# Autodesk Inventor assembly: engine moving
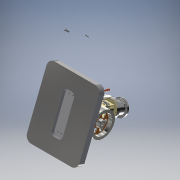
[picture p0: Inventor's stored thumbnail of the model, 180x180]
Saved by Autodesk Inventor 2017 (Build 210142000, 142)
## iProperties
Created: 2018-11-18
Part Number: engine moving
Document SubType Name: Assembly
Designer: User
Author: User
## Documents named in this file (43)
- E:\Sahil's engine\engine moving.iam
- E:\Sahil's engine\reverse gear base cast 2.ipt
- E:\Sahil's engine\reverse gear fly wheel.ipt
- E:\Sahil's engine\reverse gear crankshaft outer rod.ipt
- E:\Sahil's engine\reverse gear crankshaft counter weight 2.ipt
- E:\Sahil's engine\reverse gear crankshaft center rod.ipt
- E:\Sahil's engine\reverse gear  upper base bearing holder 1.ipt
- E:\Sahil's engine\reverse gear lower base bearing holder.ipt
- E:\Sahil's engine\reverse gear connecting rod 1.ipt
- E:\Sahil's engine\reverse gear bearing keeper.ipt
- E:\Sahil's engine\reverse gear crank rod 1.ipt
- E:\Sahil's engine\reverse gear crankrod pin 1.ipt
- E:\Sahil's engine\reverse gear cross head 1.ipt
- E:\Sahil's engine\reverse gear pistion rod.ipt
- E:\Sahil's engine\reverse gear piston.ipt
- E:\Sahil's engine\reverse gear stand.ipt
- C:\Users\User\Documents\Inventor\Content Center Files\R2017\en-US\AS 1427(03)\AS 1427 - M3 x 6(1).ipt
- E:\Sahil's engine\reverse gear standard 101.ipt
- E:\Sahil's engine\reverse gear lower cylinder cover.ipt
- E:\Sahil's engine\reverse gear cylinder.ipt
- E:\Sahil's engine\valvle plate.ipt
- E:\Sahil's engine\reverse gear steam chest.ipt
- E:\Sahil's engine\reverse gear steam chest cover.ipt
- E:\Sahil's engine\reverse gear lever ring stud.ipt
- E:\Sahil's engine\reverse gear eccentric 1.ipt
- E:\Sahil's engine\reverse gear lower trap.ipt
- E:\Sahil's engine\reverse gear trap holders.ipt
- E:\Sahil's engine\reverse gear essentric rod 2.ipt
- E:\Sahil's engine\reverse gear reverse lever ring.ipt
- E:\Sahil's engine\reverse gear blands.ipt
- E:\Sahil's engine\reverse gear steam chest rod valve 1.ipt
- E:\Sahil's engine\reverse gear steam chest side valve.ipt
- E:\Sahil's engine\reverse gear gear link.ipt
- E:\Sahil's engine\reverse gear rever lever.ipt
- C:\Users\User\Documents\Inventor\Content Center Files\R2017\en-US\AS 1427(03)\AS 1427 - M2 x 10(1).ipt
- C:\Users\User\Documents\Inventor\Content Center Files\R2017\en-US\AS 1427(03)\AS 1427 - M4 x 12(1).ipt
- E:\Sahil's engine\reverse gear link lever 1.ipt
- C:\Users\User\Documents\Inventor\Content Center Files\R2017\en-US\AS 1427(03)\AS 1427 - M3 x 16(1).ipt
- E:\Sahil's engine\reverse gear reverse gear.ipt
- E:\Sahil's engine\reverse gear link block.ipt
- E:\Sahil's engine\reverse gear drag link.ipt
- E:\Sahil's engine\reverse gear link rod.ipt
- C:\Users\User\Documents\Inventor\Content Center Files\R2017\en-US\AS 1427(01)\AS 1427 - M3.5 x 20(3).ipt
## Components (60 placed, 42 different names)
1. reverse gear fly wheel:1 — Insert:6, Mate:2, Mate:6
2. reverse gear crankshaft outer rod:1 — Insert:2, Insert:6, Mate:2, Mate:3, Insert:7, Mate:6, Mate:7, Mate:22, Rotation:1
3. reverse gear crankshaft counter weight 2:1 — Insert:2, Insert:3, Mate:7, Mate:22
4. reverse gear crankshaft counter weight 2:2 — Insert:4, Insert:5
5. reverse gear crankshaft center rod:1 — Insert:3, Insert:4, Insert:8, Rotation:1
6. reverse gear crankshaft outer rod:2 — Insert:5, Mate:3, Insert:22, Insert:23
7. reverse gear  upper base bearing holder 1:1 — Mate:4, Flush:1, Flush:2, Flush:3, Flush:4
8. reverse gear lower base bearing holder:1 — Mate:4, Flush:1, Flush:2, Insert:7, Mate:5
9. reverse gear base cast 2:1 — Mate:5, Flush:3, Flush:4, Mate:9, Flush:7, Flush:8, Flush:15, Flush:16, Mate:13, Insert:13, Insert:14, Insert:15, Insert:16, Mate:14, Flush:17, Flush:18, Insert:20, Insert:21
10. reverse gear  upper base bearing holder 1:2 — Mate:8, Flush:5, Flush:6, Flush:8
11. reverse gear lower base bearing holder:2 — Mate:8, Flush:5, Flush:6, Mate:9, Flush:7
12. reverse gear connecting rod 1:1 — Mate:10, Flush:9, Flush:10, Insert:8, Mate:12, Flush:13, Flush:14
13. reverse gear connecting rod 1:2 — Mate:10, Flush:9, Flush:10, Mate:11, Flush:11, Flush:12
14. reverse gear bearing keeper:1 — Mate:11, Flush:11, Flush:12
15. reverse gear crank rod 1:1 — Mate:12, Flush:13, Flush:14, Insert:9
16. reverse gear crankrod pin 1:1 — Insert:9, Insert:10
17. reverse gear cross head 1:1 — Insert:10, Insert:11
18. reverse gear pistion rod:1 — Insert:11, Insert:17
19. reverse gear piston:1 — Insert:17
20. reverse gear stand:1 — Flush:15, Flush:16, Mate:13
21. AS 1427 - Metric M3 x 6:1 — Insert:14
22. AS 1427 - Metric M3 x 6:2 — Insert:16
23. AS 1427 - Metric M3 x 6:3 — Insert:15
24. AS 1427 - Metric M3 x 6:4 — Insert:13
25. reverse gear standard 101:1 — Mate:14, Flush:17, Flush:18, Insert:18
26. reverse gear lower cylinder cover:1 — Insert:18, Insert:19
27. reverse gear cylinder:1 — Insert:19, Mate:15, Flush:19, Flush:20, Flush:21, Flush:22
28. valvle plate:1 — Mate:15, Flush:19, Flush:20, Mate:16
29. reverse gear steam chest:1 — Mate:16, Flush:21, Flush:22, Mate:17, Flush:23, Flush:24, Insert:29, Flush:27
30. reverse gear steam chest cover:1 — Mate:17, Flush:23, Flush:24, Mate:23
31. reverse gear lever ring stud:1 — Insert:20, Insert:28
32. reverse gear lever ring stud:2 — Insert:21, Mate:29
33. reverse gear eccentric 1:1 — Insert:22, Insert:24
34. reverse gear eccentric 1:2 — Insert:23, Insert:25
35. reverse gear lower trap:1 — Mate:20, Mate:21, Flush:26
36. reverse gear lower trap:2 — Mate:18, Mate:19, Flush:25
37. reverse gear trap holders:1 — Insert:24, Mate:18, Mate:19, Flush:25, Insert:27
38. reverse gear trap holders:2 — Insert:25, Mate:20, Mate:21, Flush:26, Insert:26
39. reverse gear essentric rod 2:1 — Insert:27, Mate:25, Mate:26
40. reverse gear essentric rod 2:2 — Insert:26, Mate:27, Mate:28
41. reverse gear reverse lever ring:1 — Insert:28, Insert:32, Insert:33, Mate:29
42. reverse gear blands:1 — Insert:29, Insert:30
43. reverse gear steam chest rod valve 1:1 — Insert:30, Insert:31, Rotation:2, Insert:43, Rotation:3
44. reverse gear steam chest side valve:1 — Insert:31, Rotation:2
45. reverse gear gear link:1 — Flush:27, Mate:23, Flush:28
46. reverse gear rever lever:1 — Insert:33, Insert:38, Mate:24
47. AS 1427 - Metric M2 x 10:3 — Insert:37, Insert:38
48. AS 1427 - Metric M2 x 10:4
49. AS 1427 - Metric M4 x 12:1 — Insert:43, Rotation:3
50. AS 1427 - Metric M4 x 12:2 — Insert:32
51. AS 1427 - Metric M4 x 12:4
52. AS 1427 - Metric M3 x 16:1 — Flush:28, Mate:24, Insert:44
53. reverse gear reverse gear:1 — Insert:40, Insert:41, Insert:42
54. reverse gear link block:1
55. reverse gear drag link:1 — Insert:37, Insert:39
56. reverse gear link rod:1 — Insert:39, Insert:40
57. AS 1427 - Metric M3.5 x 20:1 — Insert:42, Mate:27, Mate:28
58. AS 1427 - Metric M3.5 x 20:2 — Insert:41, Mate:25, Mate:26
59. reverse gear link lever 1:1
60. reverse gear link lever 1:2 — Insert:44
## Relationships (98: Insert 39, Mate 28, Flush 28, RelateRotation 3)
- Insert:2: reverse gear crankshaft outer rod:1 ↔ reverse gear crankshaft counter weight 2:1
- Insert:3 (-5 mm): reverse gear crankshaft counter weight 2:1 ↔ reverse gear crankshaft center rod:1
- Insert:4: reverse gear crankshaft counter weight 2:2 ↔ reverse gear crankshaft center rod:1
- Insert:5 (-5 mm): reverse gear crankshaft counter weight 2:2 ↔ reverse gear crankshaft outer rod:2
- Insert:6: reverse gear fly wheel:1 ↔ reverse gear crankshaft outer rod:1
- Mate:2: reverse gear fly wheel:1 ↔ reverse gear crankshaft outer rod:1
- Mate:3: reverse gear crankshaft outer rod:1 ↔ reverse gear crankshaft outer rod:2
- Mate:4: reverse gear  upper base bearing holder 1:1 ↔ reverse gear lower base bearing holder:1
- Flush:1: reverse gear  upper base bearing holder 1:1 ↔ reverse gear lower base bearing holder:1
- Flush:2 (7 mm): reverse gear  upper base bearing holder 1:1 ↔ reverse gear lower base bearing holder:1
- Insert:7 (-15 mm): reverse gear crankshaft outer rod:1 ↔ reverse gear lower base bearing holder:1
- Mate:5: reverse gear lower base bearing holder:1 ↔ reverse gear base cast 2:1
- Flush:3 (29 mm): reverse gear  upper base bearing holder 1:1 ↔ reverse gear base cast 2:1
- Flush:4: reverse gear  upper base bearing holder 1:1 ↔ reverse gear base cast 2:1
- Mate:6: reverse gear fly wheel:1 ↔ reverse gear crankshaft outer rod:1
- Mate:7: reverse gear crankshaft outer rod:1 ↔ reverse gear crankshaft counter weight 2:1
- Mate:8: reverse gear  upper base bearing holder 1:2 ↔ reverse gear lower base bearing holder:2
- Flush:5 (7 mm): reverse gear  upper base bearing holder 1:2 ↔ reverse gear lower base bearing holder:2
- Flush:6: reverse gear  upper base bearing holder 1:2 ↔ reverse gear lower base bearing holder:2
- Mate:9: reverse gear base cast 2:1 ↔ reverse gear lower base bearing holder:2
- Flush:7: reverse gear base cast 2:1 ↔ reverse gear lower base bearing holder:2
- Flush:8 (29 mm): reverse gear base cast 2:1 ↔ reverse gear  upper base bearing holder 1:2
- Mate:10: reverse gear connecting rod 1:1 ↔ reverse gear connecting rod 1:2
- Flush:9: reverse gear connecting rod 1:1 ↔ reverse gear connecting rod 1:2
- Flush:10: reverse gear connecting rod 1:1 ↔ reverse gear connecting rod 1:2
- Mate:11: reverse gear connecting rod 1:2 ↔ reverse gear bearing keeper:1
- Flush:11: reverse gear connecting rod 1:2 ↔ reverse gear bearing keeper:1
- Flush:12: reverse gear connecting rod 1:2 ↔ reverse gear bearing keeper:1
- Insert:8 (5.5 mm): reverse gear crankshaft center rod:1 ↔ reverse gear connecting rod 1:1
- Mate:12: reverse gear connecting rod 1:1 ↔ reverse gear crank rod 1:1
- Flush:13: reverse gear connecting rod 1:1 ↔ reverse gear crank rod 1:1
- Flush:14: reverse gear connecting rod 1:1 ↔ reverse gear crank rod 1:1
- Insert:9 (-14.5 mm): reverse gear crank rod 1:1 ↔ reverse gear crankrod pin 1:1
- Insert:10 (6 mm): reverse gear crankrod pin 1:1 ↔ reverse gear cross head 1:1
- Insert:11 (-8 mm): reverse gear cross head 1:1 ↔ reverse gear pistion rod:1
- Flush:15 (-58 mm): reverse gear base cast 2:1 ↔ reverse gear stand:1
- Flush:16 (53 mm): reverse gear base cast 2:1 ↔ reverse gear stand:1
- Mate:13: reverse gear base cast 2:1 ↔ reverse gear stand:1
- Insert:13 (-5.5 mm): reverse gear base cast 2:1 ↔ AS 1427 - Metric M3 x 6:4
- Insert:14 (-5.5 mm): reverse gear base cast 2:1 ↔ AS 1427 - Metric M3 x 6:1
- Insert:15 (-5.5 mm): reverse gear base cast 2:1 ↔ AS 1427 - Metric M3 x 6:3
- Insert:16 (-5.5 mm): reverse gear base cast 2:1 ↔ AS 1427 - Metric M3 x 6:2
- Mate:14: reverse gear base cast 2:1 ↔ reverse gear standard 101:1
- Flush:17: reverse gear base cast 2:1 ↔ reverse gear standard 101:1
- Flush:18 (12 mm): reverse gear base cast 2:1 ↔ reverse gear standard 101:1
- Insert:17: reverse gear pistion rod:1 ↔ reverse gear piston:1
- Insert:18 (-6.5 mm): reverse gear standard 101:1 ↔ reverse gear lower cylinder cover:1
- Insert:19: reverse gear lower cylinder cover:1 ↔ reverse gear cylinder:1
- Mate:15: reverse gear cylinder:1 ↔ valvle plate:1
- Flush:19: reverse gear cylinder:1 ↔ valvle plate:1
- Flush:20: reverse gear cylinder:1 ↔ valvle plate:1
- Mate:16: valvle plate:1 ↔ reverse gear steam chest:1
- Flush:21: reverse gear cylinder:1 ↔ reverse gear steam chest:1
- Flush:22: reverse gear cylinder:1 ↔ reverse gear steam chest:1
- Mate:17: reverse gear steam chest:1 ↔ reverse gear steam chest cover:1
- Flush:23: reverse gear steam chest:1 ↔ reverse gear steam chest cover:1
- Flush:24: reverse gear steam chest:1 ↔ reverse gear steam chest cover:1
- Insert:20 (-4.8 mm): reverse gear base cast 2:1 ↔ reverse gear lever ring stud:1
- Insert:21 (-4.8 mm): reverse gear base cast 2:1 ↔ reverse gear lever ring stud:2
- Insert:22 (-18 mm): reverse gear crankshaft outer rod:2 ↔ reverse gear eccentric 1:1
- Insert:23 (-7 mm): reverse gear crankshaft outer rod:2 ↔ reverse gear eccentric 1:2
- Insert:24: reverse gear eccentric 1:1 ↔ reverse gear trap holders:1
- Mate:18: reverse gear lower trap:2 ↔ reverse gear trap holders:1
- Mate:19: reverse gear lower trap:2 ↔ reverse gear trap holders:1
- Flush:25: reverse gear lower trap:2 ↔ reverse gear trap holders:1
- Insert:25: reverse gear eccentric 1:2 ↔ reverse gear trap holders:2
- Mate:20: reverse gear lower trap:1 ↔ reverse gear trap holders:2
- Mate:21: reverse gear lower trap:1 ↔ reverse gear trap holders:2
- Flush:26: reverse gear lower trap:1 ↔ reverse gear trap holders:2
- Insert:26 (-3.7 mm): reverse gear trap holders:2 ↔ reverse gear essentric rod 2:2
- Insert:27 (-3.7 mm): reverse gear trap holders:1 ↔ reverse gear essentric rod 2:1
- Insert:28: reverse gear lever ring stud:1 ↔ reverse gear reverse lever ring:1
- Mate:22: reverse gear crankshaft outer rod:1 ↔ reverse gear crankshaft counter weight 2:1
- Rotation:1 [RelateRotation] (1 ul): reverse gear crankshaft outer rod:1 ↔ reverse gear crankshaft center rod:1
- Insert:29 (-8 mm): reverse gear steam chest:1 ↔ reverse gear blands:1
- Insert:30 (-42 mm): reverse gear blands:1 ↔ reverse gear steam chest rod valve 1:1
- Insert:31 (-10 mm): reverse gear steam chest rod valve 1:1 ↔ reverse gear steam chest side valve:1
- Rotation:2 [RelateRotation] (1 ul): reverse gear steam chest rod valve 1:1 ↔ reverse gear steam chest side valve:1
- Flush:27 (1 mm): reverse gear steam chest:1 ↔ reverse gear gear link:1
- Mate:23: reverse gear steam chest cover:1 ↔ reverse gear gear link:1
- Insert:32: reverse gear reverse lever ring:1 ↔ AS 1427 - Metric M4 x 12:2
- Insert:33: reverse gear reverse lever ring:1 ↔ reverse gear rever lever:1
- Flush:28 (-20 mm): reverse gear gear link:1 ↔ AS 1427 - Metric M3 x 16:1
- Insert:37 (-9 mm): AS 1427 - Metric M2 x 10:3 ↔ reverse gear drag link:1
- Insert:38 (-9 mm): reverse gear rever lever:1 ↔ AS 1427 - Metric M2 x 10:3
- Insert:39 (1.9 mm): reverse gear drag link:1 ↔ reverse gear link rod:1
- Insert:40: reverse gear reverse gear:1 ↔ reverse gear link rod:1
- Mate:24: reverse gear rever lever:1 ↔ AS 1427 - Metric M3 x 16:1
- Insert:41 (-20 mm): reverse gear reverse gear:1 ↔ AS 1427 - Metric M3.5 x 20:2
- Mate:25: reverse gear essentric rod 2:1 ↔ AS 1427 - Metric M3.5 x 20:2
- Insert:42 (-20 mm): reverse gear reverse gear:1 ↔ AS 1427 - Metric M3.5 x 20:1
- Mate:26: reverse gear essentric rod 2:1 ↔ AS 1427 - Metric M3.5 x 20:2
- Mate:27: reverse gear essentric rod 2:2 ↔ AS 1427 - Metric M3.5 x 20:1
- Mate:28: reverse gear essentric rod 2:2 ↔ AS 1427 - Metric M3.5 x 20:1
- Insert:43: reverse gear steam chest rod valve 1:1 ↔ AS 1427 - Metric M4 x 12:1
- Rotation:3 [RelateRotation] (1 ul): reverse gear steam chest rod valve 1:1 ↔ AS 1427 - Metric M4 x 12:1
- Insert:44 (-6 mm): AS 1427 - Metric M3 x 16:1 ↔ reverse gear link lever 1:2
- Mate:29: reverse gear lever ring stud:2 ↔ reverse gear reverse lever ring:1
